# Autodesk Inventor assembly: Print Bed
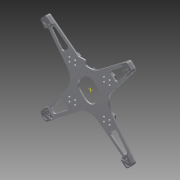
[picture p0: Inventor's stored thumbnail of the model, 180x180]
Saved by Autodesk Inventor 2014 (Build 180170000, 170)
## iProperties
Created: 2016-05-10
Part Number: Print Bed
Document SubType Name: Assembly
Designer: 101767
Author: 101767
## Documents named in this file (6)
- C:\Users\101767\Desktop\XL-print-bed\Print Bed\Print Bed.iam
- C:\Users\101767\Desktop\XL-print-bed\Print Bed\6061 Bed.ipt
- C:\Users\101767\Desktop\XL-print-bed\Print Bed\9338T520.ipt
- C:\Users\101767\Desktop\XL-print-bed\Print Bed\leveling clip.ipt
- C:\Users\101767\Desktop\XL-print-bed\Print Bed\9657K307.ipt
- C:\Users\101767\Desktop\XL-print-bed\Print Bed\90265A144.ipt
## Components (15 placed, 5 different names)
1. 6061 Bed:1 — Mate:1, Flush:1, Mate:6, Mate:7, Insert:1, Insert:2
2. 90265A144:1 — Insert:1
3. 90265A144:2 — Insert:2
4. 9338T520:1 — Mate:7, Mate:8, Flush:2
5. 9338T520:2
6. 9338T520:3
7. 9338T520:4
8. leveling clip:1 — Flush:1, Mate:5
9. 9657K307:1 — Mate:5, Mate:6
10. leveling clip:2
11. 9657K307:2
12. leveling clip:3
13. 9657K307:3
14. leveling clip:4
15. 9657K307:4
## Component patterns: Linear Bearings (4 elements), Springs and Clips (4 elements)
## Relationships (9: Mate 5, Flush 2, Insert 2)
- Mate:1: 6061 Bed:1
- Flush:1: 6061 Bed:1 ↔ leveling clip:1
- Mate:5: leveling clip:1 ↔ 9657K307:1
- Mate:6: 6061 Bed:1 ↔ 9657K307:1
- Mate:7: 6061 Bed:1 ↔ 9338T520:1
- Mate:8 (85 mm): 9338T520:1
- Flush:2 (85 mm): 9338T520:1
- Insert:1 (3 mm): 6061 Bed:1 ↔ 90265A144:1
- Insert:2 (3 mm): 6061 Bed:1 ↔ 90265A144:2
